# Autodesk Inventor assembly: Zespół1
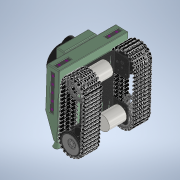
[picture p0: Inventor's stored thumbnail of the model, 180x180]
Saved by Autodesk Inventor 2022 (Build 260153000, 153)
## iProperties
Created: 2025-04-23
Part Number: Zespół1
Document SubType Name: Assembly
Designer: Olga Kowalczyk IB 240875
Author: Olga Kowalczyk IB 240875
## Documents named in this file (9)
- D:\Programy\Documents\II_EiT\ASE\ProjektCAD\Zespół1.iam
- D:\Programy\Documents\II_EiT\ASE\ProjektCAD\kolo.ipt
- D:\Programy\Documents\II_EiT\ASE\ProjektCAD\zebatka.ipt
- D:\Programy\Documents\II_EiT\ASE\ProjektCAD\silnik.ipt
- D:\Programy\Documents\II_EiT\ASE\ProjektCAD\podstawa.ipt
- D:\Programy\Documents\II_EiT\ASE\ProjektCAD\gasiennica.ipt
- D:\Programy\Documents\II_EiT\ASE\ProjektCAD\obudowa.ipt
- D:\Programy\Documents\II_EiT\ASE\ProjektCAD\led.ipt
- D:\Programy\Documents\II_EiT\ASE\ProjektCAD\lidar.ipt
## Components (29 placed, 8 different names)
1. kolo:1 — Styczny:4, Zestawiające:2, Zestawiające:3, Styczny:5
2. kolo:2 — Styczny:3, Zestawiające:1, Zestawiające:4, Styczny:6
3. silnik:1 — Wstawiające:2, Styczny:2, Wstawiające:3
4. silnik:2 — Wstawiające:1, Styczny:1, Wstawiające:4
5. podstawa:1 — Wstawiające:1, Styczny:1, Wstawiające:2, Styczny:2, Styczny:3, Zestawiające:1, Styczny:4, Zestawiające:2, Zestawiające:5
6. zebatka:1 — Wstawiające:3
7. zebatka:2 — Wstawiające:4
8. gasiennica:1 — Zestawiające:4, Styczny:6
9. gasiennica:2 — Zestawiające:3, Styczny:5
10. obudowa:1 — Zestawiające:5, Zestawiające:6, Zestawiające:7, Zestawiające:9, Zestawiające:10, Zestawiające:11, Zestawiające:12, Zestawiające:13, Zestawiające:16, Zestawiające:17, Zestawiające:28, Zestawiające:29, Zestawiające:30, Zestawiające:31, Zestawiające:32, Zestawiające:33, Zestawiające:34, Zestawiające:35, Zestawiające:36, Zestawiające:37, Zestawiające:38, Zestawiające:39, Zestawiające:40, Styczny:7
11. led:1 — Zestawiające:15, Zestawiające:16, Zestawiające:17
12. led:2 — Zestawiające:12, Zestawiające:13, Zestawiające:14, Zestawiające:15
13. led:3 — Zestawiające:8, Zestawiające:9, Zestawiające:10, Zestawiające:14
14. led:4 — Zestawiające:6, Zestawiające:7, Zestawiające:8, Zestawiające:11
15. led:5 — Zestawiające:18, Równoległe:1, Równoległe:8, Zestawiające:34
16. led:6 — Zestawiające:18, Równoległe:1, Równoległe:2, Zestawiające:19, Równoległe:6, Równoległe:8, Zestawiające:36
17. led:7 — Równoległe:2, Równoległe:3, Zestawiające:19, Zestawiające:20, Równoległe:6, Równoległe:7
18. led:8 — Równoległe:3, Równoległe:4, Zestawiające:20, Zestawiające:21, Równoległe:5, Równoległe:7
19. led:9 — Równoległe:4, Zestawiające:21, Równoległe:5, Zestawiające:35
20. led:10 — Równoległe:9, Zestawiające:22, Równoległe:16, Zestawiające:38
21. led:11 — Równoległe:9, Równoległe:10, Zestawiające:22, Zestawiające:23, Równoległe:15, Równoległe:16
22. led:12 — Równoległe:10, Równoległe:11, Zestawiające:23, Zestawiające:24, Równoległe:14, Równoległe:15
23. led:13 — Równoległe:11, Równoległe:12, Zestawiające:24, Zestawiające:25, Równoległe:13, Równoległe:14, Zestawiające:37
24. led:14 — Równoległe:12, Zestawiające:25, Równoległe:13, Zestawiające:39
25. led:15 — Równoległe:17, Zestawiające:27, Równoległe:19, Zestawiające:32, Zestawiające:33
26. led:16 — Równoległe:17, Zestawiające:27, Równoległe:19, Zestawiające:31
27. led:17 — Równoległe:18, Zestawiające:26, Równoległe:20, Zestawiające:28, Zestawiające:29, Zestawiające:30
28. led:18 — Równoległe:18, Zestawiające:26, Równoległe:20
29. lidar:1 — Zestawiające:40, Styczny:7
## Relationships (71: Mate 40, Flush 20, Tangent 7, Insert 4)
- Wstawiające:1 [Insert]: silnik:2 ↔ podstawa:1
- Styczny:1 [Tangent]: silnik:2 ↔ podstawa:1
- Wstawiające:2 [Insert]: silnik:1 ↔ podstawa:1
- Styczny:2 [Tangent]: silnik:1 ↔ podstawa:1
- Wstawiające:3 [Insert] (0.5 mm): silnik:1 ↔ zebatka:1
- Wstawiające:4 [Insert] (0.5 mm): silnik:2 ↔ zebatka:2
- Styczny:3 [Tangent]: kolo:2 ↔ podstawa:1
- Zestawiające:1 [Mate] (6 mm): kolo:2 ↔ podstawa:1
- Styczny:4 [Tangent]: kolo:1 ↔ podstawa:1
- Zestawiające:2 [Mate] (6 mm): kolo:1 ↔ podstawa:1
- Zestawiające:3 [Mate]: kolo:1 ↔ gasiennica:2
- Styczny:5 [Tangent]: kolo:1 ↔ gasiennica:2
- Zestawiające:4 [Mate]: kolo:2 ↔ gasiennica:1
- Styczny:6 [Tangent]: kolo:2 ↔ gasiennica:1
- Zestawiające:5 [Mate] (9 mm): podstawa:1 ↔ obudowa:1
- Zestawiające:6 [Mate]: obudowa:1 ↔ led:4
- Zestawiające:7 [Mate]: obudowa:1 ↔ led:4
- Zestawiające:8 [Mate]: led:3 ↔ led:4
- Zestawiające:9 [Mate]: obudowa:1 ↔ led:3
- Zestawiające:10 [Mate]: obudowa:1 ↔ led:3
- Zestawiające:11 [Mate]: obudowa:1 ↔ led:4
- Zestawiające:12 [Mate]: obudowa:1 ↔ led:2
- Zestawiające:13 [Mate]: obudowa:1 ↔ led:2
- Zestawiające:14 [Mate]: led:2 ↔ led:3
- Zestawiające:15 [Mate]: led:1 ↔ led:2
- Zestawiające:16 [Mate]: obudowa:1 ↔ led:1
- Zestawiające:17 [Mate]: obudowa:1 ↔ led:1
- Zestawiające:18 [Mate]: led:5 ↔ led:6
- Równoległe:1 [Flush]: led:5 ↔ led:6
- Równoległe:2 [Flush]: led:6 ↔ led:7
- Równoległe:3 [Flush]: led:7 ↔ led:8
- Równoległe:4 [Flush]: led:8 ↔ led:9
- Zestawiające:19 [Mate]: led:6 ↔ led:7
- Zestawiające:20 [Mate]: led:7 ↔ led:8
- Zestawiające:21 [Mate]: led:8 ↔ led:9
- Równoległe:5 [Flush]: led:8 ↔ led:9
- Równoległe:6 [Flush]: led:6 ↔ led:7
- Równoległe:7 [Flush]: led:7 ↔ led:8
- Równoległe:8 [Flush]: led:5 ↔ led:6
- Równoległe:9 [Flush]: led:10 ↔ led:11
- Równoległe:10 [Flush]: led:11 ↔ led:12
- Równoległe:11 [Flush]: led:12 ↔ led:13
- Równoległe:12 [Flush]: led:13 ↔ led:14
- Zestawiające:22 [Mate]: led:10 ↔ led:11
- Zestawiające:23 [Mate]: led:11 ↔ led:12
- Zestawiające:24 [Mate]: led:12 ↔ led:13
- Zestawiające:25 [Mate]: led:13 ↔ led:14
- Równoległe:13 [Flush]: led:13 ↔ led:14
- Równoległe:14 [Flush]: led:12 ↔ led:13
- Równoległe:15 [Flush]: led:11 ↔ led:12
- Równoległe:16 [Flush]: led:10 ↔ led:11
- Równoległe:17 [Flush]: led:15 ↔ led:16
- Równoległe:18 [Flush]: led:17 ↔ led:18
- Zestawiające:26 [Mate]: led:17 ↔ led:18
- Zestawiające:27 [Mate]: led:15 ↔ led:16
- Równoległe:19 [Flush]: led:15 ↔ led:16
- Równoległe:20 [Flush]: led:17 ↔ led:18
- Zestawiające:28 [Mate]: obudowa:1 ↔ led:17
- Zestawiające:29 [Mate]: obudowa:1 ↔ led:17
- Zestawiające:30 [Mate]: obudowa:1 ↔ led:17
- Zestawiające:31 [Mate]: obudowa:1 ↔ led:16
- Zestawiające:32 [Mate]: obudowa:1 ↔ led:15
- Zestawiające:33 [Mate]: obudowa:1 ↔ led:15
- Zestawiające:34 [Mate]: obudowa:1 ↔ led:5
- Zestawiające:35 [Mate]: obudowa:1 ↔ led:9
- Zestawiające:36 [Mate]: obudowa:1 ↔ led:6
- Zestawiające:37 [Mate]: obudowa:1 ↔ led:13
- Zestawiające:38 [Mate]: obudowa:1 ↔ led:10
- Zestawiające:39 [Mate]: obudowa:1 ↔ led:14
- Zestawiające:40 [Mate]: obudowa:1 ↔ lidar:1
- Styczny:7 [Tangent] (2.5 mm): obudowa:1 ↔ lidar:1
